# Autodesk Inventor assembly: ShooterFrameAssembly05
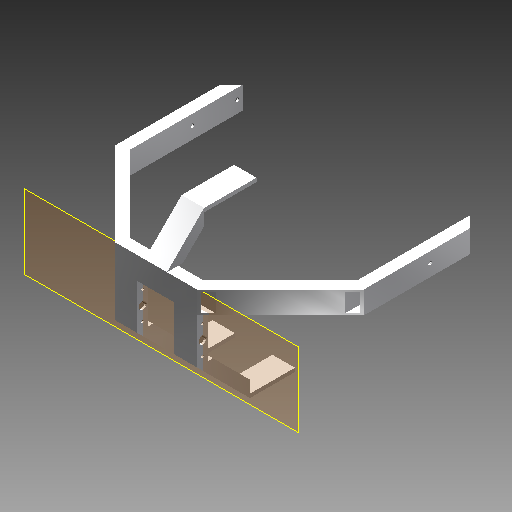
[picture p0: Inventor's stored thumbnail of the model, 512x512]
Saved by Autodesk Inventor 2017 SP1 (Build 210196100, 196)
## iProperties
Created: 2016-02-08
Part Number: ShooterFrameAssembly05
Document SubType Name: Assembly
Designer: steele
Author: steele
## Documents named in this file (6)
- D:\snobotics\CAD-Development\robSteele\SnoBotics2016\2016-05-05-ShooterPrototype\ShooterFrameAssembly05.iam
- D:\snobotics\CAD-Development\robSteele\SnoBotics2016\2016-05-05-ShooterPrototype\ShooterFrameV02.ipt
- D:\snobotics\CAD-Development\robSteele\SnoBotics2016\2016-05-05-ShooterPrototype\45dege0_75x1.50.ipt
- D:\snobotics\CAD-Development\robSteele\SnoBotics2016\2016-05-05-ShooterPrototype\bottomOfShooter.ipt
- D:\snobotics\CAD-Development\robSteele\SnoBotics2016\2016-05-05-ShooterPrototype\45dege0_75x1.50ForTopOfShooter.ipt
- D:\snobotics\CAD-Development\robSteele\SnoBotics2016\2016-05-05-ShooterPrototype\topOfShooter.ipt
## Components (7 placed, 5 different names)
1. ShooterFrameV02:1 — Mate:1, Mate:2, Mate:3, Mate:4, Flush:10, Mate:9, Mate:10, Mate:11
2. 45dege0_75x1.50:1 — Mate:1, Mate:2, Mate:5, Mate:6
3. 45dege0_75x1.50:2 — Mate:3, Mate:4, Mate:7, Mate:8
4. bottomOfShooter:1 — Mate:5, Mate:6, Flush:2
5. bottomOfShooter:2 — Mate:7, Mate:8, Flush:2
6. 45dege0_75x1.50ForTopOfShooter:1 — Flush:10, Mate:9, Mate:10, Mate:12, Mate:13
7. topOfShooter:1 — Mate:11, Mate:12, Mate:13
## Relationships (16: Mate 13, Flush 3)
- Flush:1 (160.3502 mm)
- Mate:1: ShooterFrameV02:1 ↔ 45dege0_75x1.50:1
- Mate:2: ShooterFrameV02:1 ↔ 45dege0_75x1.50:1
- Mate:3: ShooterFrameV02:1 ↔ 45dege0_75x1.50:2
- Mate:4: ShooterFrameV02:1 ↔ 45dege0_75x1.50:2
- Mate:5: 45dege0_75x1.50:1 ↔ bottomOfShooter:1
- Mate:6: 45dege0_75x1.50:1 ↔ bottomOfShooter:1
- Mate:7: 45dege0_75x1.50:2 ↔ bottomOfShooter:2
- Mate:8: 45dege0_75x1.50:2 ↔ bottomOfShooter:2
- Flush:2: bottomOfShooter:1 ↔ bottomOfShooter:2
- Flush:10: ShooterFrameV02:1 ↔ 45dege0_75x1.50ForTopOfShooter:1
- Mate:9: ShooterFrameV02:1 ↔ 45dege0_75x1.50ForTopOfShooter:1
- Mate:10: ShooterFrameV02:1 ↔ 45dege0_75x1.50ForTopOfShooter:1
- Mate:11: ShooterFrameV02:1 ↔ topOfShooter:1
- Mate:12: 45dege0_75x1.50ForTopOfShooter:1 ↔ topOfShooter:1
- Mate:13: 45dege0_75x1.50ForTopOfShooter:1 ↔ topOfShooter:1
